# Autodesk Inventor assembly: RR
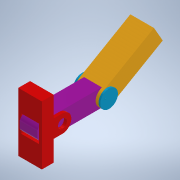
[picture p0: Inventor's stored thumbnail of the model, 180x180]
Saved by Autodesk Inventor 2021 (Build 250183000, 183)
## iProperties
Created: 2022-04-29
Part Number: RR
Document SubType Name: Assembly
Designer: Administrator
Title: Solution v2
Author: Administrator
## Documents named in this file (5)
- C:\Users\youss\OneDrive\Desktop\PRNEW\PR.iam
- C:\Users\youss\OneDrive\Desktop\PRNEW\Base v3.ipt
- C:\Users\youss\OneDrive\Desktop\PRNEW\Motor v2.ipt
- C:\Users\youss\OneDrive\Desktop\PRNEW\End v2.ipt
- C:\Users\youss\OneDrive\Desktop\PRNEW\Middle v2.ipt
## Components (4 placed, 4 different names)
1. Base v3:1 — Slider:1
2. Motor v2:2 — Rigid:2, Rotational:2
3. End v2:1 — Rigid:2
4. Middle v2:1 — Rotational:2, Slider:1
## Relationships (3: WeldJoint 1, RevoluteJoint 1, TranslationJoint 1)
- Rigid:2 [WeldJoint]: Motor v2:2 ↔ End v2:1
- Rotational:2 [RevoluteJoint]: Motor v2:2 ↔ Middle v2:1
- Slider:1 [TranslationJoint]: Base v3:1 ↔ Middle v2:1
